# Autodesk Inventor assembly: Cơ cấu gạt cốc
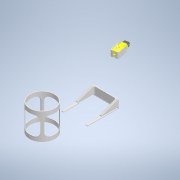
[picture p0: Inventor's stored thumbnail of the model, 180x180]
Saved by Autodesk Inventor 2020 (Build 240168000, 168)
## iProperties
Created: 2022-04-01
Part Number: Cơ cấu gạt cốc
Document SubType Name: Assembly
Designer: PC
Author: PC
## Documents named in this file (6)
- D:\Do-an-tot-nghiep\Cơ cấu gạt cốc.iam
- D:\Do-an-tot-nghiep\Hộp đựng động cơ.ipt
- D:\Do-an-tot-nghiep\Khay đựng cốc.ipt
- D:\Do-an-tot-nghiep\Khay gạt cốc.ipt
- D:\Do-an-tot-nghiep\Thanh đẩy khay gạt.ipt
- C:\Users\PC\Downloads\motor-box.ipt
## Components (5 placed, 5 different names)
1. Hộp đựng động cơ:1 — Mate:1, Mate:2, Mate:3, Mate:4
2. Khay đựng cốc:1
3. Khay gạt cốc:1
4. Thanh đẩy khay gạt:1
5. motor-box:1 — Mate:1, Mate:2, Mate:3, Mate:4
## Relationships (4: Mate 4)
- Mate:1: Hộp đựng động cơ:1 ↔ motor-box:1
- Mate:2: Hộp đựng động cơ:1 ↔ motor-box:1
- Mate:3: Hộp đựng động cơ:1 ↔ motor-box:1
- Mate:4: Hộp đựng động cơ:1 ↔ motor-box:1
